# Autodesk Inventor assembly: EnsamblajeSwitch
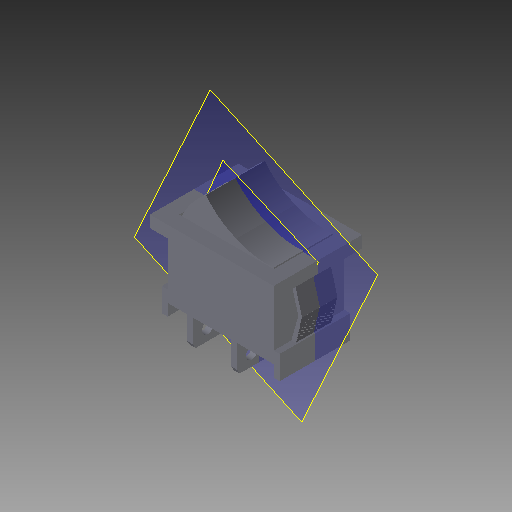
[picture p0: Inventor's stored thumbnail of the model, 512x512]
Saved by Autodesk Inventor 2017 (Build 210142000, 142)
## iProperties
Created: 2016-05-14
Part Number: EnsamblajeSwitch
Document SubType Name: Assembly
Designer: Isra
Author: Isra
## Documents named in this file (6)
- C:\Users\franc\Desktop\EsialRobotik\Mecanique\composants\Interrupteur\Switch simple\EnsamblajeSwitch.iam
- C:\Users\franc\Desktop\EsialRobotik\Mecanique\composants\Interrupteur\Switch simple\Base.ipt
- C:\Users\franc\Desktop\EsialRobotik\Mecanique\composants\Interrupteur\Switch simple\Polo2.ipt
- C:\Users\franc\Desktop\EsialRobotik\Mecanique\composants\Interrupteur\Switch simple\Pieza2.ipt
- C:\Users\franc\Desktop\EsialRobotik\Mecanique\composants\Interrupteur\Switch simple\Sw.ipt
- C:\Users\franc\Desktop\EsialRobotik\Mecanique\composants\Interrupteur\Switch simple\InteriorSw.ipt
## Components (5 placed, 5 different names)
1. Base:1 — Nivelación:1, Nivelación:2, Coincidencia:1, Coincidencia:2, Simetría:1
2. Polo2:1 — Nivelación:1, Nivelación:4, Nivelación:5
3. Pieza2:1 — Nivelación:2
4. Sw:1 — Coincidencia:1, Coincidencia:2, Simetría:1, Tangente:1
5. InteriorSw:1 — Nivelación:4, Tangente:1, Nivelación:5
## Relationships (8: Flush 4, Mate 2, Symmetry 1, Tangent 1)
- Nivelación:1 [Flush]: Base:1 ↔ Polo2:1
- Nivelación:2 [Flush]: Base:1 ↔ Pieza2:1
- Coincidencia:1 [Mate]: Base:1 ↔ Sw:1
- Coincidencia:2 [Mate]: Base:1 ↔ Sw:1
- Simetría:1 [Symmetry]: Base:1 ↔ Sw:1
- Nivelación:4 [Flush]: Polo2:1 ↔ InteriorSw:1
- Tangente:1 (-2 mm): Sw:1 ↔ InteriorSw:1
- Nivelación:5 [Flush] (1 mm): Polo2:1 ↔ InteriorSw:1
